# Autodesk Inventor assembly: Light Holder
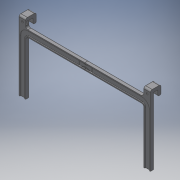
[picture p0: Inventor's stored thumbnail of the model, 180x180]
Saved by Autodesk Inventor 2017 (Build 210142000, 142)
## iProperties
Created: 2017-03-25
Part Number: Light Holder
Document SubType Name: Assembly
Designer: Diego
Author: Diego
## Documents named in this file (4)
- C:\Users\Alex\Dropbox\Arduino\arduinoLED_BGLighting\Hardware\Light Holder.iam
- C:\Users\Alex\Dropbox\Arduino\arduinoLED_BGLighting\Hardware\Top Clip.ipt
- C:\Users\Alex\Dropbox\Arduino\arduinoLED_BGLighting\Hardware\Top Clip_MIR.ipt
- C:\Users\Alex\Dropbox\Arduino\arduinoLED_BGLighting\Hardware\Bow Tie Key.ipt
## Components (3 placed, 3 different names)
1. Top Clip:1 — Flush:1, Flush:2
2. Top Clip_MIR:1
3. Bow Tie Key:1 — Flush:1, Flush:2
## Relationships (2: Flush 2)
- Flush:1: Top Clip:1 ↔ Bow Tie Key:1
- Flush:2: Top Clip:1 ↔ Bow Tie Key:1
